# Autodesk Inventor assembly: tukurikake
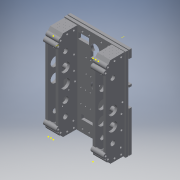
[picture p0: Inventor's stored thumbnail of the model, 180x180]
Saved by Autodesk Inventor 2018 (Build 220112000, 112)
## iProperties
Created: 2018-08-16
Part Number: tukurikake
Material: 一般
Document SubType Name: Assembly
Designer: shun2
Author: shun2
## Documents named in this file (4)
- C:\Users\shun2\OneDrive\おそらく最新版(2018.7.31)\ギアボックス\tukurikake.iam
- C:\Users\shun2\OneDrive\おそらく最新版(2018.7.31)\ギアボックス\ギアボックス片側.iam
- C:\Users\shun2\OneDrive\おそらく最新版(2018.7.31)\1枚目\一枚目.ipt
- C:\Users\shun2\OneDrive\おそらく最新版(2018.7.31)\2枚目\2枚目.ipt
## Components (4 placed, 3 different names)
1. ギアボックス片側:1 [sub-assembly]
2. ギアボックス片側:2 [sub-assembly]
3. 一枚目:1 — メイト:1, メイト:3
4. 2枚目:1 — メイト:2, メイト:4
## Relationships (4: Mate 4)
- メイト:1 [Mate]: 一枚目:1
- メイト:2 [Mate]: 2枚目:1
- メイト:3 [Mate]: 一枚目:1
- メイト:4 [Mate]: 2枚目:1
